# Autodesk Inventor assembly: Belt_Unit_Asem_Rev2
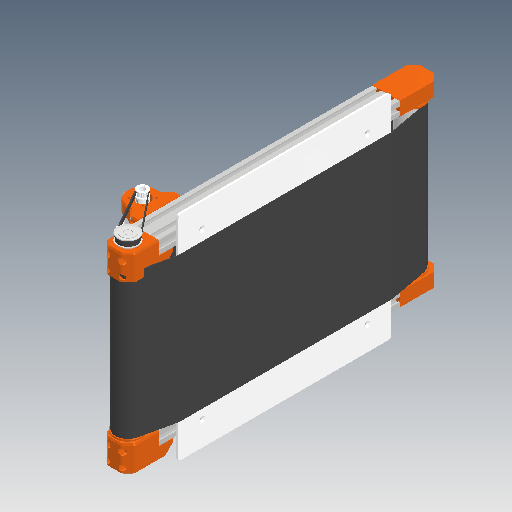
[picture p0: Inventor's stored thumbnail of the model, 512x512]
Saved by Autodesk Inventor 2020.1 (Build 241239000, 239)
## iProperties
Created: 2020-10-05
Part Number: Belt_Unit_Asem_Rev2
Document SubType Name: Assembly
Designer: kenta iguchi
Author: kenta iguchi
## Documents named in this file (19)
- D:\ken113\Documents\GitHub\Cheap_Belt_Printer\Model\Asem\Belt_Unit_Asem_Rev2.iam
- D:\ken113\Documents\GitHub\Cheap_Belt_Printer\Model\Parts\Bed_Parts\Bed Plate.ipt
- D:\ken113\Documents\GitHub\Cheap_Belt_Printer\Model\Parts\Stepper Motor\NEMA17\Nema17_Geard\NEMA17_Geard.iam
- D:\ken113\Documents\GitHub\Cheap_Belt_Printer\Model\Parts\Print_Parts\Print_Parts_K.ipt
- D:\ken113\Documents\GitHub\Cheap_Belt_Printer\Model\Parts\MISUMI\FL6900ZZ_Autodesk_Inventor_2020_20201006\FL6900ZZ.ipt
- D:\ken113\Documents\GitHub\Cheap_Belt_Printer\Model\Parts\Print_Parts\Print_Parts_L.ipt
- D:\ken113\Documents\GitHub\Cheap_Belt_Printer\Model\Parts\Print_Parts\Print_Parts_N.ipt
- D:\ken113\Documents\GitHub\Cheap_Belt_Printer\Model\Parts\Pulley\GT2\GT2_20t\GT2_20teeth_8bore.ipt
- D:\ken113\Documents\GitHub\Cheap_Belt_Printer\Model\Parts\MISUMI\GPA40GT2060-A-H10_Autodesk_Inventor_2020_20201006\AIS2020\GPA40GT2060-A-H10_b.ipt
- D:\ken113\Documents\GitHub\Cheap_Belt_Printer\Model\Parts\Print_Parts\Print_Parts_O.ipt
- D:\ken113\Documents\GitHub\Cheap_Belt_Printer\Model\Parts\Shop_Parts\Φ35mm_Pipe.ipt
- D:\ken113\Documents\GitHub\Cheap_Belt_Printer\Model\Parts\Print_Parts\Print_Parts_P.ipt
- D:\ken113\Documents\GitHub\Cheap_Belt_Printer\Model\Parts\Print_Parts\Print_Parts_Q.ipt
- D:\ken113\Documents\GitHub\Cheap_Belt_Printer\Model\Parts\Print_Parts\Print_Parts_R.ipt
- D:\ken113\Documents\GitHub\Cheap_Belt_Printer\Model\Parts\MISUMI\SSFRW10-230-MD6-N6_Autodesk_Inventor_2020_20201006\AIS2020\SSFRW10-230-MD6-N6_s.ipt
- D:\ken113\Documents\GitHub\Cheap_Belt_Printer\Model\Parts\MISUMI\SSFR10-280_Autodesk_Inventor_2020_20201006\AIS2020\SSFR10-280_s.ipt
- D:\ken113\Documents\GitHub\Cheap_Belt_Printer\Model\Parts\MISUMI\HFS5-2040-350_Autodesk_Inventor_2020_20201006\HFS5-2040-350.ipt
- D:\ken113\Documents\GitHub\Cheap_Belt_Printer\Model\Parts\Bed_Parts\Build_Belt.ipt
- D:\ken113\Documents\GitHub\Cheap_Belt_Printer\Model\Parts\Bed_Parts\Bed_Unit_Belt.ipt
## Components (31 placed, 18 different names)
1. Bed Plate:1 — メイト:13
2. Φ35mm_Pipe:1 — メイト:14, 挿入:22
3. Print_Parts_K:1 — フラッシュ:25
4. Print_Parts_K:2
5. Φ35mm_Pipe:2 — 挿入:23
6. Print_Parts_P:2 — フラッシュ:25
7. Print_Parts_P:1
8. FL6900ZZ:3 — 挿入:17
9. FL6900ZZ:4
10. HFS5-2040-350:1 — メイト:24, フラッシュ:29, フラッシュ:30
11. NEMA17_Geard:2 [sub-assembly] — メイト:17, メイト:19, 挿入:16, メイト:20
12. Print_Parts_L:1 — フラッシュ:21, メイト:13, 挿入:9, 挿入:10, メイト:14, メイト:15
13. HFS5-2040-350:2
14. Print_Parts_L:2 — フラッシュ:21, 挿入:12, 挿入:13, 挿入:14, メイト:16, フラッシュ:26, フラッシュ:27, メイト:21
15. FL6900ZZ:5 — 挿入:9, 挿入:11
16. FL6900ZZ:6 — 挿入:10, 挿入:15
17. Print_Parts_N:1 — メイト:15, 挿入:11
18. FL6900ZZ:7 — 挿入:12
19. FL6900ZZ:8 — 挿入:13
20. Print_Parts_N:2 — 挿入:14, メイト:16
21. GT2_20teeth_8bore:1 — メイト:17, フラッシュ:23, メイト:26
22. GPA40GT2060-A-H10_b:1 — 挿入:15, フラッシュ:23, 挿入:21, 挿入:24
23. Print_Parts_O:1 — メイト:19, 挿入:16, メイト:20
24. Print_Parts_R:1 — 挿入:17, 挿入:19, フラッシュ:28, メイト:22, メイト:23
25. SSFRW10-230-MD6-N6_s:1 — 挿入:19, 挿入:20
26. Print_Parts_R:2 — 挿入:20, フラッシュ:28, メイト:25
27. Print_Parts_Q:1 — フラッシュ:26, フラッシュ:27, メイト:21, メイト:22, メイト:23
28. SSFR10-280_s:1 — 挿入:21
29. Print_Parts_Q:2 — メイト:24, フラッシュ:29, フラッシュ:30, メイト:25
30. Build_Belt:1 — 挿入:22, 挿入:23
31. Bed_Unit_Belt:1 — 挿入:24, メイト:26
## Relationships (56: Insert 21, Mate 18, Flush 16, Angle 1)
- [Insert]: Φ35mm_Pipe:1 ↔ Print_Parts_K:1
- [Insert]: Φ35mm_Pipe:1 ↔ Print_Parts_K:2
- [Insert]: Φ35mm_Pipe:2 ↔ Print_Parts_P:2
- [Insert]: Φ35mm_Pipe:2 ↔ Print_Parts_P:1
- [Insert]: Print_Parts_P:2 ↔ FL6900ZZ:3
- [Insert]: Print_Parts_P:1 ↔ FL6900ZZ:4
- [Mate] (5 mm): Bed Plate:1 ↔ HFS5-2040-350:1
- [Flush] (25 mm): Bed Plate:1 ↔ HFS5-2040-350:1
- [Mate]: HFS5-2040-350:1 ↔ Print_Parts_L:1
- [Flush]: HFS5-2040-350:1 ↔ Print_Parts_L:1
- [Flush]: HFS5-2040-350:1 ↔ Print_Parts_L:1
- [Mate] (2 mm): Print_Parts_K:2 ↔ HFS5-2040-350:1
- [Mate]: HFS5-2040-350:2 ↔ Print_Parts_L:2
- [Flush]: HFS5-2040-350:2 ↔ Print_Parts_L:2
- [Flush]: HFS5-2040-350:2 ↔ Print_Parts_L:2
- [Flush]: HFS5-2040-350:1 ↔ HFS5-2040-350:2
- フラッシュ:21 [Flush]: Print_Parts_L:1 ↔ Print_Parts_L:2
- [Flush] (-25 mm): Bed Plate:1 ↔ HFS5-2040-350:2
- メイト:13 [Mate] (20 mm): Bed Plate:1 ↔ Print_Parts_L:1
- 挿入:9 [Insert]: Print_Parts_L:1 ↔ FL6900ZZ:5
- 挿入:10 [Insert]: Print_Parts_L:1 ↔ FL6900ZZ:6
- メイト:14 [Mate]: Φ35mm_Pipe:1 ↔ Print_Parts_L:1
- メイト:15 [Mate]: Print_Parts_L:1 ↔ Print_Parts_N:1
- 挿入:11 [Insert]: FL6900ZZ:5 ↔ Print_Parts_N:1
- 挿入:12 [Insert]: Print_Parts_L:2 ↔ FL6900ZZ:7
- 挿入:13 [Insert]: Print_Parts_L:2 ↔ FL6900ZZ:8
- 挿入:14 [Insert]: Print_Parts_L:2 ↔ Print_Parts_N:2
- メイト:16 [Mate]: Print_Parts_L:2 ↔ Print_Parts_N:2
- メイト:17 [Mate]: NEMA17_Geard:2 ↔ GT2_20teeth_8bore:1
- 挿入:15 [Insert] (0.5 mm): FL6900ZZ:6 ↔ GPA40GT2060-A-H10_b:1
- フラッシュ:23 [Flush]: GT2_20teeth_8bore:1 ↔ GPA40GT2060-A-H10_b:1
- [Mate]: HFS5-2040-350:1 ↔ Print_Parts_O:1
- [Flush]: HFS5-2040-350:1 ↔ Print_Parts_O:1
- メイト:19 [Mate]: NEMA17_Geard:2 ↔ Print_Parts_O:1
- 挿入:16 [Insert]: NEMA17_Geard:2 ↔ Print_Parts_O:1
- メイト:20 [Mate]: NEMA17_Geard:2 ↔ Print_Parts_O:1
- フラッシュ:25 [Flush]: Print_Parts_K:1 ↔ Print_Parts_P:2
- 挿入:17 [Insert] (0.5 mm): FL6900ZZ:3 ↔ Print_Parts_R:1
- 挿入:19 [Insert] (-5 mm): Print_Parts_R:1 ↔ SSFRW10-230-MD6-N6_s:1
- 挿入:20 [Insert]: SSFRW10-230-MD6-N6_s:1 ↔ Print_Parts_R:2
- フラッシュ:26 [Flush]: Print_Parts_L:2 ↔ Print_Parts_Q:1
- フラッシュ:27 [Flush]: Print_Parts_L:2 ↔ Print_Parts_Q:1
- メイト:21 [Mate] (350 mm): Print_Parts_L:2 ↔ Print_Parts_Q:1
- フラッシュ:28 [Flush]: Print_Parts_R:1 ↔ Print_Parts_R:2
- [Angle] (0 deg): HFS5-2040-350:1 ↔ Print_Parts_R:1
- メイト:22 [Mate]: Print_Parts_R:1 ↔ Print_Parts_Q:1
- メイト:23 [Mate]: Print_Parts_R:1 ↔ Print_Parts_Q:1
- 挿入:21 [Insert]: GPA40GT2060-A-H10_b:1 ↔ SSFR10-280_s:1
- メイト:24 [Mate]: HFS5-2040-350:1 ↔ Print_Parts_Q:2
- フラッシュ:29 [Flush]: HFS5-2040-350:1 ↔ Print_Parts_Q:2
- フラッシュ:30 [Flush]: HFS5-2040-350:1 ↔ Print_Parts_Q:2
- メイト:25 [Mate] (5 mm): Print_Parts_R:2 ↔ Print_Parts_Q:2
- 挿入:22 [Insert]: Φ35mm_Pipe:1 ↔ Build_Belt:1
- 挿入:23 [Insert]: Φ35mm_Pipe:2 ↔ Build_Belt:1
- 挿入:24 [Insert]: GPA40GT2060-A-H10_b:1 ↔ Bed_Unit_Belt:1
- メイト:26 [Mate]: GT2_20teeth_8bore:1 ↔ Bed_Unit_Belt:1
## Named parameters: d60_d54 = 0 mm, d61_d55 = 0 mm, d62_d56 = 0 mm, d63_d57 = 0 mm, d43_d37 = 0 mm, d44_d38 = 0 mm, d45_d39 = 0 mm
